# Autodesk Inventor assembly: 2.75 Omni Assembly
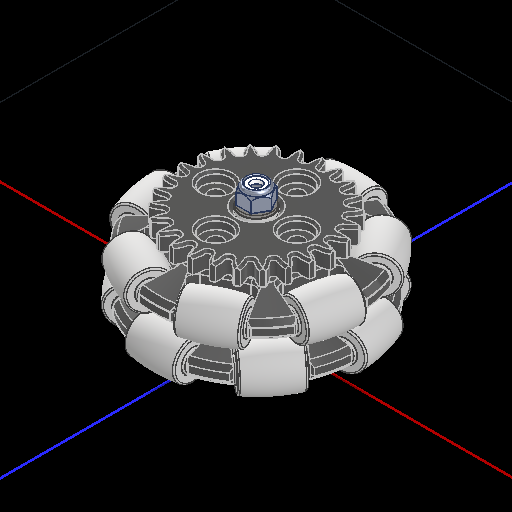
[picture p0: Inventor's stored thumbnail of the model, 512x512]
Saved by Autodesk Inventor 2025.2 (Build 292293000, 293)
## iProperties
Created: 2025-11-15
Part Number: 2.75 Omni Assembly
Document SubType Name: Assembly
Designer: cloudy
Author: cloudy
## Documents named in this file (11)
- C:\Users\cloudy\Documents\AURA_CAD\15\Drivetrain\Wheels\Omni\2.75\2.75 Omni Assembly.iam
- C:\Users\cloudy\Documents\AURA_CAD\15\Drivetrain\Wheels\Omni\2.75\2.75 inner.ipt
- C:\Users\cloudy\Documents\AURA_CAD\15\Drivetrain\Wheels\Omni\2.75\2.75 nut outer.ipt
- C:\Users\cloudy\Documents\AURA_CAD\15\Drivetrain\Wheels\Omni\2.75\2.75 outer no nut.ipt
- C:\Users\cloudy\Documents\AURA_CAD\!lib\Motion\4 inch omni roller.ipt
- C:\Users\cloudy\Documents\AURA_CAD\!lib\Motion\Insert Circle.ipt
- C:\Users\cloudy\Documents\AURA_CAD\!lib\Structure\Hardware\Nut Hex.ipt
- C:\Users\cloudy\Documents\AURA_CAD\15\Drivetrain\Gears\26t.ipt
- C:\Users\cloudy\Documents\AURA_CAD\!lib\Motion\Spacers\Washer Steel\SWasher .375 OD x .031250.ipt
- C:\Users\cloudy\Documents\AURA_CAD\!lib\Motion\Spacers\Washer Steel.ipt
- C:\Users\cloudy\Documents\AURA_CAD\!lib\Structure\Hardware\Nut Nylock.ipt
## Components (28 placed, 9 different names)
1. 2.75 inner:1 — Insert:1, Mate:1, Mate:3, Tangent:3, Tangent:4, Mate:5, Insert:7
2. 2.75 nut outer:1 — Mate:3, Insert:6, Insert:7, Insert:8, Insert:9, Insert:10, Insert:11
3. 2.75 outer no nut:1 — Mate:2, Insert:4, Insert:12
4. 2.75 inner:2 — Insert:1, Mate:1, Mate:2, Tangent:1, Tangent:2, Mate:4, Insert:4
5. Insert Circle:2 — Insert:6, Insert:14
6. Nut Hex:1 — Insert:9
7. Nut Hex:2 — Insert:10
8. Nut Hex:3 — Insert:8
9. Nut Hex:4 — Insert:11
10. 26t:1 — Insert:12, Insert:13
11. Insert Circle:3 — Insert:13, Insert:15
12. SWasher .375 OD x .031250:1 — Insert:14
13. SWasher .375 OD x .031250:2 — Insert:15, Insert:16
14. Nut Nylock:1 — Insert:16
15. 4 inch omni roller:1 — Tangent:1, Tangent:2, Mate:4
16. 4 inch omni roller:2 — Tangent:3, Tangent:4, Mate:5
17. 4 inch omni roller:3
18. 4 inch omni roller:4
19. 4 inch omni roller:5
20. 4 inch omni roller:6
21. 4 inch omni roller:7
22. 4 inch omni roller:8
23. 4 inch omni roller:9
24. 4 inch omni roller:10
25. 4 inch omni roller:11
26. 4 inch omni roller:12
27. 4 inch omni roller:13
28. 4 inch omni roller:14
## Component patterns: (7 elements, first: 4 inch omni roller:1 + 4 inch omni roller:2)
## Relationships (22: Insert 13, Mate 5, Tangent 4)
- Insert:1: 2.75 inner:1 ↔ 2.75 inner:2
- Mate:1: 2.75 inner:1 ↔ 2.75 inner:2
- Mate:2: 2.75 outer no nut:1 ↔ 2.75 inner:2
- Mate:3: 2.75 inner:1 ↔ 2.75 nut outer:1
- Tangent:1: 2.75 inner:2 ↔ 4 inch omni roller:1
- Tangent:2: 2.75 inner:2 ↔ 4 inch omni roller:1
- Mate:4 (0.25 mm): 2.75 inner:2 ↔ 4 inch omni roller:1
- Tangent:3: 2.75 inner:1 ↔ 4 inch omni roller:2
- Tangent:4: 2.75 inner:1 ↔ 4 inch omni roller:2
- Mate:5 (0.25 mm): 2.75 inner:1 ↔ 4 inch omni roller:2
- Insert:4: 2.75 outer no nut:1 ↔ 2.75 inner:2
- Insert:6: 2.75 nut outer:1 ↔ Insert Circle:2
- Insert:7: 2.75 inner:1 ↔ 2.75 nut outer:1
- Insert:8: 2.75 nut outer:1 ↔ Nut Hex:3
- Insert:9: 2.75 nut outer:1 ↔ Nut Hex:1
- Insert:10: 2.75 nut outer:1 ↔ Nut Hex:2
- Insert:11: 2.75 nut outer:1 ↔ Nut Hex:4
- Insert:12: 2.75 outer no nut:1 ↔ 26t:1
- Insert:13: 26t:1 ↔ Insert Circle:3
- Insert:14: Insert Circle:2 ↔ SWasher .375 OD x .031250:1
- Insert:15: Insert Circle:3 ↔ SWasher .375 OD x .031250:2
- Insert:16: SWasher .375 OD x .031250:2 ↔ Nut Nylock:1
